# Autodesk Inventor assembly: Extender
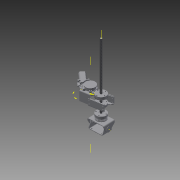
[picture p0: Inventor's stored thumbnail of the model, 180x180]
Saved by Autodesk Inventor 2013 (Build 170138000, 138)
## iProperties
Created: 2013-01-18
Part Number: Extender
Document SubType Name: Assembly
Designer: actoennies
Mass: 1580.93 g
Surface Area: 2717.1 cm^2
Volume: 641.09 cm^3
Density: 2.466 g/cm^3
Author: actoennies
## Documents named in this file (16)
- \\NNHSSRV2.hs.sd203.org\ACToennies$\Robotics\Shooter\Extender.iam
- \\NNHSSRV2.hs.sd203.org\ACToennies$\Robotics\Shooter\Flange.ipt
- \\NNHSSRV2.hs.sd203.org\ACToennies$\Robotics\Shooter\ACME Threaded Rod Nut.ipt
- \\NNHSSRV2.hs.sd203.org\ACToennies$\Robotics\Shooter\Hub 2.ipt
- \\NNHSSRV2.hs.sd203.org\ACToennies$\Robotics\Shooter\Spacer Plate 2.ipt
- \\NNHSSRV2.hs.sd203.org\ACToennies$\Robotics\Shooter\Bearing.ipt
- \\NNHSSRV2.hs.sd203.org\ACToennies$\Robotics\Shooter\ASME Threaded Rod.ipt
- \\NNHSSRV2.hs.sd203.org\ACToennies$\Robotics\Shooter\Bearing Mount 4 v1.ipt
- \\NNHSSRV2.hs.sd203.org\ACToennies$\Robotics\Shooter\Short Hex Shaft.ipt
- \\NNHSSRV2.hs.sd203.org\ACToennies$\Robotics\Shooter\Bearing Mount 5.ipt
- \\NNHSSRV2.hs.sd203.org\ACToennies$\Robotics\Shooter\Bearing Mount 3 v1.ipt
- H:\Robotics\Parts\Imported Components\Snow Blower Motor\Snow Blower Motor.iam
- \\NNHSSRV2.hs.sd203.org\ACToennies$\Robotics\Shooter\Snow Blower Hub.ipt
- \\NNHSSRV2.hs.sd203.org\ACToennies$\Robotics\Shooter\Gear for Extender.ipt
- \\NNHSSRV2.hs.sd203.org\ACToennies$\Robotics\Shooter\Gear for Extender 2.ipt
- \\NNHSSRV2.hs.sd203.org\ACToennies$\Robotics\Shooter\Snowblower Motor Mount.ipt
## Components (28 placed, 15 different names)
1. Flange:1 — Insert:1, Insert:2, Insert:3
2. ACME Threaded Rod Nut:1 — Insert:1, Insert:8
3. Hub 2:1 — Insert:2, Insert:3, Insert:4, Insert:5
4. Spacer Plate 2:1 — Insert:4, Insert:5, Insert:6, Insert:7, Insert:9
5. Hub 2:2 — Insert:6, Insert:7
6. ASME Threaded Rod:1 — Insert:8, Mate:8, Mate:12, Mate:18, Mate:21
7. Bearing:1 — Insert:9, Mate:9, Mate:10, Insert:13
8. Bearing Mount 4 v1:1 — Insert:10, Insert:11, Insert:12, Angle:1
9. Bearing:2 — Insert:12, Insert:13, Mate:11
10. Bearing:3 — Insert:11, Flush:2, Mate:6, Mate:7, Insert:14
11. Bearing:4 — Insert:10, Flush:1, Mate:4, Mate:5, Insert:15
12. Short Hex Shaft:1 — Flush:1, Mate:4, Mate:5, Flush:3
13. Short Hex Shaft:2 — Flush:2, Mate:6, Mate:7, Flush:3
14. Short Hex Shaft:3 — Mate:8, Mate:9, Mate:10, Mate:11
15. Bearing:5 — Insert:14
16. Bearing:6 — Insert:15, Insert:16
17. Bearing Mount 5:1 — Insert:16, Angle:1
18. ACME Threaded Rod Nut:2 — Mate:12, Insert:17
19. Flange:2 — Insert:17, Insert:18, Insert:19, Insert:20, Insert:21
20. Bearing Mount 3 v1:1 — Insert:18, Insert:19, Angle:2, Mate:22
21. Bearing Mount 3 v1:2 — Insert:20, Insert:21
22. Snow Blower Motor:1 [sub-assembly] — Mate:13, Mate:14, Mate:16, Mate:17, Mate:20, Insert:26, Insert:27
23. Snow Blower Hub:1 — Mate:13, Mate:14, Mate:15, Mate:17, Flush:4, Mate:19, Insert:25
24. ACME Threaded Rod Nut:3 — Insert:22, Mate:18
25. Flange:3 — Insert:22, Insert:23, Insert:24, Flush:4
26. Gear for Extender:1 — Insert:23, Insert:24
27. Gear for Extender 2:1 — Mate:19, Insert:25
28. Snowblower Motor Mount:1 — Insert:26, Insert:27, Angle:2, Mate:22
## Relationships (52: Insert 27, Mate 19, Flush 4, Angle 2)
- Insert:1: Flange:1 ↔ ACME Threaded Rod Nut:1
- Insert:2: Flange:1 ↔ Hub 2:1
- Insert:3: Flange:1 ↔ Hub 2:1
- Insert:4: Hub 2:1 ↔ Spacer Plate 2:1
- Insert:5: Hub 2:1 ↔ Spacer Plate 2:1
- Insert:6: Spacer Plate 2:1 ↔ Hub 2:2
- Insert:7: Spacer Plate 2:1 ↔ Hub 2:2
- Insert:8: ACME Threaded Rod Nut:1 ↔ ASME Threaded Rod:1
- Insert:9: Spacer Plate 2:1 ↔ Bearing:1
- Insert:10: Bearing Mount 4 v1:1 ↔ Bearing:4
- Insert:11: Bearing Mount 4 v1:1 ↔ Bearing:3
- Insert:12: Bearing Mount 4 v1:1 ↔ Bearing:2
- Flush:1: Bearing:4 ↔ Short Hex Shaft:1
- Mate:4: Bearing:4 ↔ Short Hex Shaft:1
- Mate:5: Bearing:4 ↔ Short Hex Shaft:1
- Flush:2: Bearing:3 ↔ Short Hex Shaft:2
- Mate:6: Bearing:3 ↔ Short Hex Shaft:2
- Mate:7: Bearing:3 ↔ Short Hex Shaft:2
- Flush:3: Short Hex Shaft:1 ↔ Short Hex Shaft:2
- Mate:8 (3.175 mm): ASME Threaded Rod:1 ↔ Short Hex Shaft:3
- Mate:9: Bearing:1 ↔ Short Hex Shaft:3
- Mate:10: Bearing:1 ↔ Short Hex Shaft:3
- Insert:13 (3.175 mm): Bearing:1 ↔ Bearing:2
- Mate:11: Bearing:2 ↔ Short Hex Shaft:3
- Insert:14: Bearing:3 ↔ Bearing:5
- Insert:15: Bearing:4 ↔ Bearing:6
- Insert:16: Bearing:6 ↔ Bearing Mount 5:1
- Angle:1 (0 deg): Bearing Mount 4 v1:1 ↔ Bearing Mount 5:1
- Mate:12: ASME Threaded Rod:1 ↔ ACME Threaded Rod Nut:2
- Insert:17: ACME Threaded Rod Nut:2 ↔ Flange:2
- Insert:18: Flange:2 ↔ Bearing Mount 3 v1:1
- Insert:19: Flange:2 ↔ Bearing Mount 3 v1:1
- Insert:20: Flange:2 ↔ Bearing Mount 3 v1:2
- Insert:21: Flange:2 ↔ Bearing Mount 3 v1:2
- Mate:13: Snow Blower Motor:1 ↔ Snow Blower Hub:1
- Mate:14: Snow Blower Motor:1 ↔ Snow Blower Hub:1
- Mate:15: Snow Blower Hub:1
- Mate:16: Snow Blower Motor:1
- Mate:17: Snow Blower Motor:1 ↔ Snow Blower Hub:1
- Insert:22: ACME Threaded Rod Nut:3 ↔ Flange:3
- Mate:18: ASME Threaded Rod:1 ↔ ACME Threaded Rod Nut:3
- Insert:23: Flange:3 ↔ Gear for Extender:1
- Insert:24: Flange:3 ↔ Gear for Extender:1
- Flush:4: Snow Blower Hub:1 ↔ Flange:3
- Mate:19: Snow Blower Hub:1 ↔ Gear for Extender 2:1
- Insert:25: Snow Blower Hub:1 ↔ Gear for Extender 2:1
- Mate:20: Snow Blower Motor:1
- Mate:21 (63.5 mm): ASME Threaded Rod:1
- Insert:26: Snow Blower Motor:1 ↔ Snowblower Motor Mount:1
- Insert:27: Snow Blower Motor:1 ↔ Snowblower Motor Mount:1
- Angle:2 (180 deg): Bearing Mount 3 v1:1 ↔ Snowblower Motor Mount:1
- Mate:22: Bearing Mount 3 v1:1 ↔ Snowblower Motor Mount:1
